# Autodesk Inventor assembly: (FINAL)rollerAssembly
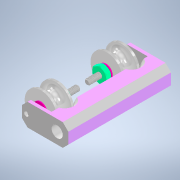
[picture p0: Inventor's stored thumbnail of the model, 180x180]
Saved by Autodesk Inventor 2022 (Build 260153000, 153)
## iProperties
Created: 2022-11-15
Part Number: (FINAL)rollerAssembly
Document SubType Name: Assembly
Designer: matia
Author: matia
## Documents named in this file (7)
- C:\Users\natha\Documents\GitHub\RelativityProjUMD\(V2) FULL ASSEMBLY\(FINAL)rollerAssembly.iam
- C:\Users\natha\Documents\GitHub\RelativityProjUMD\(V2) FULL ASSEMBLY\rollerbase(v2).ipt
- C:\Users\natha\Documents\GitHub\RelativityProjUMD\(V2) FULL ASSEMBLY\92949A333_18-8 Stainless Steel Button Head Hex Drive Screw.ipt
- C:\Users\natha\Documents\GitHub\RelativityProjUMD\(V2) FULL ASSEMBLY\wheel.ipt
- C:\Users\natha\Documents\GitHub\RelativityProjUMD\(V2) FULL ASSEMBLY\wheelbushing.ipt
- C:\Users\natha\Documents\GitHub\RelativityProjUMD\(V2) FULL ASSEMBLY\rollerwasher.ipt
- C:\Users\natha\Documents\GitHub\RelativityProjUMD\(V2) FULL ASSEMBLY\90480A006_Low-Strength Steel Hex Nut (.125).ipt
## Components (13 placed, 6 different names)
1. rollerbase(v2):1
2. 92949A333_18-8 Stainless Steel Button Head Hex Drive Screw:1 — Mate:15, Mate:16, Mate:19, Mate:20, Mate:22
3. 92949A333_18-8 Stainless Steel Button Head Hex Drive Screw:2 — Mate:17, Mate:18, Mate:21
4. wheel:1 — Mate:11, Mate:12
5. wheel:2 — Mate:13, Mate:14
6. wheelbushing:1 — Mate:11, Mate:12, Mate:16
7. wheelbushing:2 — Mate:13, Mate:14, Mate:15
8. rollerwasher:1 — Mate:17
9. rollerwasher:2 — Mate:18
10. rollerwasher:3 — Mate:19
11. rollerwasher:4 — Mate:20
12. 90480A006_Low-Strength Steel Hex Nut (.125):1 — Mate:21
13. 90480A006_Low-Strength Steel Hex Nut (.125):2 — Mate:22
## Relationships (12: Mate 12)
- Mate:11: wheel:1 ↔ wheelbushing:1
- Mate:12: wheel:1 ↔ wheelbushing:1
- Mate:13: wheel:2 ↔ wheelbushing:2
- Mate:14: wheel:2 ↔ wheelbushing:2
- Mate:15: 92949A333_18-8 Stainless Steel Button Head Hex Drive Screw:1 ↔ wheelbushing:2
- Mate:16: 92949A333_18-8 Stainless Steel Button Head Hex Drive Screw:1 ↔ wheelbushing:1
- Mate:17: 92949A333_18-8 Stainless Steel Button Head Hex Drive Screw:2 ↔ rollerwasher:1
- Mate:18: 92949A333_18-8 Stainless Steel Button Head Hex Drive Screw:2 ↔ rollerwasher:2
- Mate:19: 92949A333_18-8 Stainless Steel Button Head Hex Drive Screw:1 ↔ rollerwasher:3
- Mate:20: 92949A333_18-8 Stainless Steel Button Head Hex Drive Screw:1 ↔ rollerwasher:4
- Mate:21: 92949A333_18-8 Stainless Steel Button Head Hex Drive Screw:2 ↔ 90480A006_Low-Strength Steel Hex Nut (.125):1
- Mate:22: 92949A333_18-8 Stainless Steel Button Head Hex Drive Screw:1 ↔ 90480A006_Low-Strength Steel Hex Nut (.125):2
